# Autodesk Inventor assembly: 45mm wheel(with sleeve)
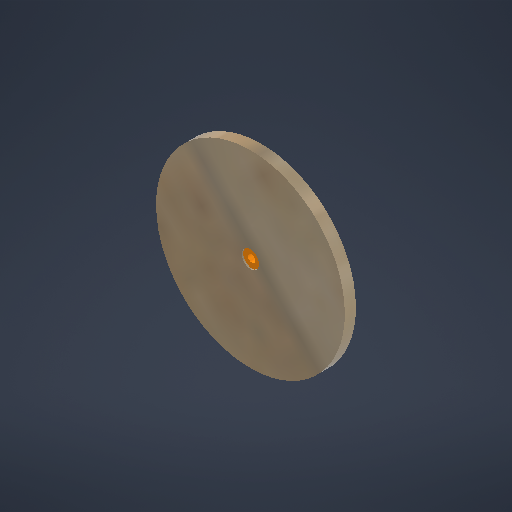
[picture p0: Inventor's stored thumbnail of the model, 512x512]
Saved by Autodesk Inventor 2025.3 (Build 293356030, 356C)
## iProperties
Created: 2025-09-05
Part Number: 45mm wheel(with sleeve)
Document SubType Name: Assembly
Designer: 陳泓任
Author: 陳泓任
## Documents named in this file (3)
- C:\Users\Ou918\3D-model-temp\introduction to mechanical engineering(1)\51mm wheel(with sleeve).iam
- C:\Users\Ou918\3D-model-temp\introduction to mechanical engineering(1)\51mm wheel.ipt
- C:\Users\Ou918\3D-model-temp\introduction to mechanical engineering(1)\sleeve.ipt
## Components (2 placed, 2 different names)
1. 51mm wheel:1 — 插入:1, 貼合:2
2. sleeve:1 — 插入:1, 貼合:1
## Relationships (3: Mate 2, Insert 1)
- 插入:1 [Insert]: 51mm wheel:1 ↔ sleeve:1
- 貼合:1 [Mate]: sleeve:1
- 貼合:2 [Mate] (-1.5 mm): 51mm wheel:1
